# Autodesk Inventor assembly: IMA+47AhFoMoCo
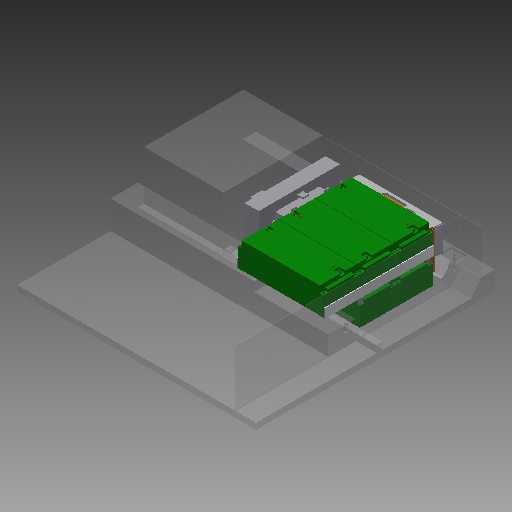
[picture p0: Inventor's stored thumbnail of the model, 512x512]
Saved by Autodesk Inventor 2017 (Build 210142000, 142)
## iProperties
Created: 2022-08-13
Part Number: IMA+47AhFoMoCo
Document SubType Name: Assembly
Designer: JTS
Author: JTS
## Documents named in this file (11)
- C:\Users\Windermac\Desktop\MASTER Honda Insight G1 IMA Bay\01 IMA+47AhFoMoCo (Pre-Tray).iam
- C:\Users\Windermac\Desktop\MASTER Honda Insight G1 IMA Bay\OEM Parts\IMA Bay - Battery Enclosure Interface.ipt
- C:\Users\Windermac\Desktop\MASTER Honda Insight G1 IMA Bay\Battery Modules\47Ah-FoMoCo.ipt
- C:\Users\Windermac\Desktop\MASTER Honda Insight G1 IMA Bay\OEM Parts\IMA Battery Case Primitive.ipt
- C:\Users\Windermac\Desktop\MASTER Honda Insight G1 IMA Bay\LiBCM PCB\LiBCM Safety Cover - RevC.ipt
- C:\Users\Windermac\Desktop\MASTER Honda Insight G1 IMA Bay\OEM Parts\Junction Board.ipt
- C:\Users\Windermac\Desktop\MASTER Honda Insight G1 IMA Bay\LiBCM004 - Battery Rail\Bracket - 5th Module 8982K875.ipt
- C:\Users\Windermac\Desktop\MASTER Honda Insight G1 IMA Bay\Battery Modules\Top Lithium Modules.iam
- C:\Users\Windermac\Desktop\MASTER Honda Insight G1 IMA Bay\LiBCM PCB\PCB.ipt
- C:\Users\Windermac\Desktop\MASTER Honda Insight G1 IMA Bay\OEM Parts\MCM.ipt
- C:\Users\Windermac\Desktop\MASTER Honda Insight G1 IMA Bay\Nuts & Bolts\Threaded Standoff.ipt
## Components (15 placed, 10 different names)
1. IMA Bay - Battery Enclosure Interface:1 — Mate:1, Flush:1, Mate:2, Insert:6, Angle:1, Mate:34, Mate:38, Mate:40, Mate:41, Mate:43
2. IMA Battery Case Primitive:1 — Insert:6, Angle:1, Insert:7, Insert:8, Mate:47
3. LiBCM Safety Cover - RevC:1 — Insert:31, Mate:39, Mate:40, Mate:41, Mate:47
4. PCB:1 — Insert:31, Mate:39
5. Bracket - 5th Module:1 — Insert:45, Insert:46
6. Top Lithium Modules:1 [sub-assembly] — Flush:38, Insert:49
7. Bracket - 5th Module:2 — Mate:48, Insert:47, Insert:48, Insert:49
8. Threaded Standoff:2 — Insert:42, Insert:47
9. Threaded Standoff:5 — Insert:43, Insert:46
10. Threaded Standoff:7 — Insert:41, Insert:48
11. Threaded Standoff:8 — Insert:44, Insert:45
12. 47Ah-FoMoCo:14 — Mate:38, Mate:42, Flush:36, Insert:41, Insert:44
13. 47Ah-FoMoCo:16 — Mate:34, Mate:42, Flush:36, Mate:43, Flush:40, Insert:42, Insert:43
14. Junction Board:1 — Insert:7, Insert:8
15. MCM:2 — Flush:38, Flush:40, Mate:48
## Relationships (30: Insert 13, Mate 11, Flush 5, Angle 1)
- Mate:1: IMA Bay - Battery Enclosure Interface:1
- Flush:1: IMA Bay - Battery Enclosure Interface:1
- Mate:2: IMA Bay - Battery Enclosure Interface:1
- Insert:6: IMA Bay - Battery Enclosure Interface:1 ↔ IMA Battery Case Primitive:1
- Angle:1 (180 deg): IMA Bay - Battery Enclosure Interface:1 ↔ IMA Battery Case Primitive:1
- [Flush]: 47Ah-FoMoCo:14 ↔ 47Ah-FoMoCo:16
- Mate:34 (3 mm): IMA Bay - Battery Enclosure Interface:1 ↔ 47Ah-FoMoCo:16
- Insert:7: IMA Battery Case Primitive:1 ↔ Junction Board:1
- Insert:8: IMA Battery Case Primitive:1 ↔ Junction Board:1
- Mate:38 (35 mm): IMA Bay - Battery Enclosure Interface:1 ↔ 47Ah-FoMoCo:14
- Insert:31 (37 mm): LiBCM Safety Cover - RevC:1 ↔ PCB:1
- Mate:39: LiBCM Safety Cover - RevC:1 ↔ PCB:1
- Mate:40 (5 mm): IMA Bay - Battery Enclosure Interface:1 ↔ LiBCM Safety Cover - RevC:1
- Mate:41 (31.5 mm): IMA Bay - Battery Enclosure Interface:1 ↔ LiBCM Safety Cover - RevC:1
- Mate:42 (2 mm): 47Ah-FoMoCo:14 ↔ 47Ah-FoMoCo:16
- Flush:36: 47Ah-FoMoCo:14 ↔ 47Ah-FoMoCo:16
- Mate:43 (28 mm): IMA Bay - Battery Enclosure Interface:1 ↔ 47Ah-FoMoCo:16
- Mate:47 (10 mm): IMA Battery Case Primitive:1 ↔ LiBCM Safety Cover - RevC:1
- Flush:38 (-8 mm): Top Lithium Modules:1 ↔ MCM:2
- Flush:40 (6 mm): 47Ah-FoMoCo:16 ↔ MCM:2
- Mate:48 (5 mm): Bracket - 5th Module:2 ↔ MCM:2
- Insert:41: Threaded Standoff:7 ↔ 47Ah-FoMoCo:14
- Insert:42: Threaded Standoff:2 ↔ 47Ah-FoMoCo:16
- Insert:43: Threaded Standoff:5 ↔ 47Ah-FoMoCo:16
- Insert:44: Threaded Standoff:8 ↔ 47Ah-FoMoCo:14
- Insert:45: Bracket - 5th Module:1 ↔ Threaded Standoff:8
- Insert:46: Bracket - 5th Module:1 ↔ Threaded Standoff:5
- Insert:47: Bracket - 5th Module:2 ↔ Threaded Standoff:2
- Insert:48: Bracket - 5th Module:2 ↔ Threaded Standoff:7
- Insert:49: Top Lithium Modules:1 ↔ Bracket - 5th Module:2
## Named parameters: d77_d35 = 0 mm
